# Autodesk Inventor assembly: 組合1
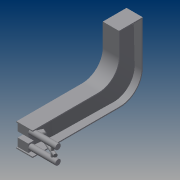
[picture p0: Inventor's stored thumbnail of the model, 180x180]
Saved by Autodesk Inventor 2018 (Build 220112000, 112)
## iProperties
Created: 2020-12-31
Part Number: 組合1
Material: 一般
Document SubType Name: Assembly
Designer: 88697
Author: 88697
## Documents named in this file (5)
- C:\Users\88697\Desktop\高爾夫球\組合1.iam
- C:\Users\88697\Desktop\高爾夫球\軌道.ipt
- C:\Users\88697\Desktop\高爾夫球\旋轉軸.ipt
- C:\Users\88697\Desktop\高爾夫球\槌子.ipt
- C:\Users\88697\Desktop\高爾夫球\槌子支架.ipt
## Components (4 placed, 4 different names)
1. 軌道:1 — 貼合:1, 齊平:1, 相切:1, 貼合:5
2. 旋轉軸:1 — 貼合:2, 貼合:3, 貼合:4
3. 槌子:1 — 貼合:4, 貼合:5
4. 槌子支架:1 — 貼合:1, 齊平:1, 相切:1, 貼合:2, 貼合:3
## Relationships (7: Mate 5, Flush 1, Tangent 1)
- 貼合:1 [Mate]: 軌道:1 ↔ 槌子支架:1
- 齊平:1 [Flush]: 軌道:1 ↔ 槌子支架:1
- 相切:1 [Tangent]: 軌道:1 ↔ 槌子支架:1
- 貼合:2 [Mate]: 旋轉軸:1 ↔ 槌子支架:1
- 貼合:3 [Mate]: 旋轉軸:1 ↔ 槌子支架:1
- 貼合:4 [Mate]: 旋轉軸:1 ↔ 槌子:1
- 貼合:5 [Mate]: 軌道:1 ↔ 槌子:1
